# Autodesk Inventor assembly: P16-5M-09AL
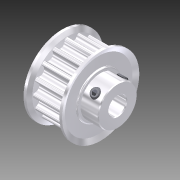
[picture p0: Inventor's stored thumbnail of the model, 180x180]
Saved by Autodesk Inventor 2011 (Build 150239000, 239)
## iProperties
Category: Miscellaneous
Company: Autodesk Inc.
Created: 2008-12-06
Part Number: P16-5M-09AL
Document SubType Name: Assembly
Designer: Autodesk Inc.
Catalog Web Link: http://www.gates.com/catalogs/file_display.cfm?file=SynchronousMetal.pdf&thisPath=gates\catalogs
Description: Sprocket 16 tooth
Vendor: Gates
Mass: 18.144 g
Surface Area: 38.6109 cm^2
Volume: 5.69952 cm^3
Author: Autodesk Inc.
## Documents named in this file (3)
- R:\2012\Inventor\vkop\All_Miscellaneous\SupportingSprocket_Gates_P16-5M-09AL.iam
- R:\2012\Inventor\vkop\All_Miscellaneous\SupportingSprocket_Gates_P16-5M-09AL.ipt
- R:\2012\Inventor\vkop\All_Miscellaneous\ANSI B18.3 - 6-32 UNC - 0.19(24).ipt
## Components (3 placed, 2 different names)
1. SupportingSprocket_Gates_P16-5M-09AL:1 — Mate:1, Mate:2
2. Hexagon Socket Set Screw - Flat Point - Inch 6-32 UNC x 0.19:1 — Mate:1
3. Hexagon Socket Set Screw - Flat Point - Inch 6-32 UNC x 0.19:2 — Mate:2
## Relationships (2: Mate 2)
- Mate:1: SupportingSprocket_Gates_P16-5M-09AL:1 ↔ Hexagon Socket Set Screw - Flat Point - Inch 6-32 UNC x 0.19:1
- Mate:2: SupportingSprocket_Gates_P16-5M-09AL:1 ↔ Hexagon Socket Set Screw - Flat Point - Inch 6-32 UNC x 0.19:2
